# Autodesk Inventor assembly: Assembly2
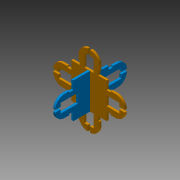
[picture p0: Inventor's stored thumbnail of the model, 180x180]
Saved by Autodesk Inventor 2014 (Build 180170000, 170)
## iProperties
Created: 2014-11-24
Part Number: Assembly2
Document SubType Name: Assembly
Designer: JLM
Author: JLM
## Documents named in this file (3)
- C:\Users\JLM\Documents\Puzzle Box\BSizeBox\Assembly2.iam
- C:\Users\JLM\Documents\Puzzle Box\BSizeBox\LockX.ipt
- C:\Users\JLM\Documents\Puzzle Box\BSizeBox\LockZ.ipt
## Components (2 placed, 2 different names)
1. LockX:1 — Mate:3, Mate:4, Flush:1
2. LockZ:1 — Mate:3, Mate:4, Flush:1
## Relationships (3: Mate 2, Flush 1)
- Mate:3: LockX:1 ↔ LockZ:1
- Mate:4: LockX:1 ↔ LockZ:1
- Flush:1: LockX:1 ↔ LockZ:1
